# Autodesk Inventor assembly: Shooter
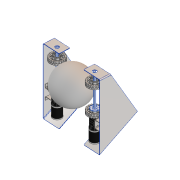
[picture p0: Inventor's stored thumbnail of the model, 180x180]
Saved by Autodesk Inventor 2016 (Build 200138000, 138)
## iProperties
Created: 2016-01-25
Part Number: Shooter
Document SubType Name: Assembly
Designer: CAD
Author: CAD
## Documents named in this file (9)
- C:\Users\PrashantBIA\Desktop\Robotics\Robot Assembly 1-27-15 New Swami\Robot Assembly\Shooter\Shooter.iam
- C:\Users\PrashantBIA\Desktop\Robotics\Robot Assembly 1-27-15 New Swami\Robot Assembly\Shooter\Imported Components\4 in HiGrip Wheel\4 in HiGrip Wheel.iam
- C:\Users\PrashantBIA\Desktop\Robotics\Robot Assembly 1-27-15 New Swami\Robot Assembly\Shooter\VersaPlanetaryWithCim.iam
- C:\Users\PrashantBIA\Desktop\Robotics\Robot Assembly 1-27-15 New Swami\Robot Assembly\Shooter\Ball.ipt
- C:\Users\PrashantBIA\Desktop\Robotics\Robot Assembly 1-27-15 New Swami\Robot Assembly\Shooter\Imported Components\am-0096a+500+Hex+Hub+r2\am-0096a+500+Hex+Hub+r2.ipt
- C:\Users\PrashantBIA\Desktop\Robotics\Robot Assembly 1-27-15 New Swami\Robot Assembly\Shooter\10inshaft.ipt
- C:\Users\PrashantBIA\Desktop\Robotics\Robot Assembly 1-27-15 New Swami\Robot Assembly\Shooter\RightMounting.ipt
- C:\Users\PrashantBIA\Desktop\Robotics\Robot Assembly 1-27-15 New Swami\Robot Assembly\Shooter\MountingForGearbox.ipt
- C:\Users\PrashantBIA\Desktop\Robotics\Robot Assembly 1-27-15 New Swami\Robot Assembly\Shooter\LeftMounting.ipt
## Components (19 placed, 8 different names)
1. VersaPlanetaryWithCim:1 [sub-assembly] — Mate:5, Flush:3, Mate:44, Flush:4, Angle:4, Angle:8, Angle:9, Mate:78, Mate:81, Mate:82
2. VersaPlanetaryWithCim:2 [sub-assembly] — Mate:2, Mate:3, Flush:3, Mate:44, Flush:4, Angle:1, Mate:52, Mate:62, Mate:84, Mate:86, Mate:87
3. Ball:1
4. 10inshaft:1 — Mate:70, Angle:7, Mate:75, Mate:76, Angle:8, Flush:8
5. 10inshaft:2 — Angle:5, Angle:6, Mate:61, Mate:62, Mate:63, Flush:9
6. RightMounting:1 — Angle:9, Mate:78, Flush:8, Mate:79
7. MountingForGearbox:1 — Mate:81, Mate:82
8. LeftMounting:1 — Mate:83, Flush:9, Mate:84, Mate:85
9. MountingForGearbox:2 — Mate:85, Mate:86, Mate:87
10. am-0096a+500+Hex+Hub+r2:1 — Mate:58, Mate:59, Mate:60, Angle:4, Mate:70
11. am-0096a+500+Hex+Hub+r2:2 — Mate:49, Mate:50, Mate:51, Angle:5, Angle:6, Mate:61, Mate:63, Flush:5, Flush:6, Mate:83
12. am-0096a+500+Hex+Hub+r2:3 — Mate:46, Mate:47, Mate:48, Angle:1, Mate:52
13. am-0096a+500+Hex+Hub+r2:4 — Mate:71, Mate:72, Mate:73, Mate:79
14. am-0096a+500+Hex+Hub+r2:5 — Mate:64, Mate:65, Mate:66, Angle:7, Mate:75, Mate:76
15. am-0096a+500+Hex+Hub+r2:7 — Mate:67, Mate:68, Mate:69, Flush:5, Flush:6
16. 4 in HiGrip Wheel:1 [sub-assembly] — Flush:1, Mate:5, Mate:58, Mate:59, Mate:60, Mate:71, Mate:72, Mate:73, Mate:74
17. 4 in HiGrip Wheel:2 [sub-assembly] — Flush:1, Mate:2, Mate:3, Mate:46, Mate:47, Mate:48, Mate:49, Mate:50, Mate:51, Mate:77
18. 4 in HiGrip Wheel:3 [sub-assembly] — Mate:64, Mate:65, Mate:66, Mate:74, Flush:7
19. 4 in HiGrip Wheel:4 [sub-assembly] — Mate:67, Mate:68, Mate:69, Mate:77, Flush:7
## Relationships (55: Mate 40, Flush 8, Angle 7)
- Flush:1: 4 in HiGrip Wheel:1 ↔ 4 in HiGrip Wheel:2
- Mate:2: VersaPlanetaryWithCim:2 ↔ 4 in HiGrip Wheel:2
- Mate:3: VersaPlanetaryWithCim:2 ↔ 4 in HiGrip Wheel:2
- Mate:5: VersaPlanetaryWithCim:1 ↔ 4 in HiGrip Wheel:1
- Flush:3: VersaPlanetaryWithCim:1 ↔ VersaPlanetaryWithCim:2
- Mate:44 (254 mm): VersaPlanetaryWithCim:1 ↔ VersaPlanetaryWithCim:2
- Flush:4: VersaPlanetaryWithCim:1 ↔ VersaPlanetaryWithCim:2
- Mate:46: am-0096a+500+Hex+Hub+r2:3 ↔ 4 in HiGrip Wheel:2
- Mate:47: am-0096a+500+Hex+Hub+r2:3 ↔ 4 in HiGrip Wheel:2
- Mate:48: am-0096a+500+Hex+Hub+r2:3 ↔ 4 in HiGrip Wheel:2
- Mate:49: am-0096a+500+Hex+Hub+r2:2 ↔ 4 in HiGrip Wheel:2
- Mate:50: am-0096a+500+Hex+Hub+r2:2 ↔ 4 in HiGrip Wheel:2
- Mate:51: am-0096a+500+Hex+Hub+r2:2 ↔ 4 in HiGrip Wheel:2
- Angle:1 (0 deg): VersaPlanetaryWithCim:2 ↔ am-0096a+500+Hex+Hub+r2:3
- Mate:52: VersaPlanetaryWithCim:2 ↔ am-0096a+500+Hex+Hub+r2:3
- Mate:58: am-0096a+500+Hex+Hub+r2:1 ↔ 4 in HiGrip Wheel:1
- Mate:59: am-0096a+500+Hex+Hub+r2:1 ↔ 4 in HiGrip Wheel:1
- Mate:60: am-0096a+500+Hex+Hub+r2:1 ↔ 4 in HiGrip Wheel:1
- Angle:4 (0 deg): VersaPlanetaryWithCim:1 ↔ am-0096a+500+Hex+Hub+r2:1
- Angle:5 (0 deg): 10inshaft:2 ↔ am-0096a+500+Hex+Hub+r2:2
- Angle:6 (0 deg): 10inshaft:2 ↔ am-0096a+500+Hex+Hub+r2:2
- Mate:61: 10inshaft:2 ↔ am-0096a+500+Hex+Hub+r2:2
- Mate:62: VersaPlanetaryWithCim:2 ↔ 10inshaft:2
- Mate:63: 10inshaft:2 ↔ am-0096a+500+Hex+Hub+r2:2
- Mate:64: am-0096a+500+Hex+Hub+r2:5 ↔ 4 in HiGrip Wheel:3
- Mate:65: am-0096a+500+Hex+Hub+r2:5 ↔ 4 in HiGrip Wheel:3
- Mate:66: am-0096a+500+Hex+Hub+r2:5 ↔ 4 in HiGrip Wheel:3
- Mate:67: am-0096a+500+Hex+Hub+r2:7 ↔ 4 in HiGrip Wheel:4
- Mate:68: am-0096a+500+Hex+Hub+r2:7 ↔ 4 in HiGrip Wheel:4
- Mate:69: am-0096a+500+Hex+Hub+r2:7 ↔ 4 in HiGrip Wheel:4
- Mate:70: 10inshaft:1 ↔ am-0096a+500+Hex+Hub+r2:1
- Mate:71: am-0096a+500+Hex+Hub+r2:4 ↔ 4 in HiGrip Wheel:1
- Mate:72: am-0096a+500+Hex+Hub+r2:4 ↔ 4 in HiGrip Wheel:1
- Mate:73: am-0096a+500+Hex+Hub+r2:4 ↔ 4 in HiGrip Wheel:1
- Mate:74: 4 in HiGrip Wheel:1 ↔ 4 in HiGrip Wheel:3
- Angle:7 (0 deg): 10inshaft:1 ↔ am-0096a+500+Hex+Hub+r2:5
- Mate:75: 10inshaft:1 ↔ am-0096a+500+Hex+Hub+r2:5
- Mate:76: 10inshaft:1 ↔ am-0096a+500+Hex+Hub+r2:5
- Angle:8 (0 deg): VersaPlanetaryWithCim:1 ↔ 10inshaft:1
- Mate:77: 4 in HiGrip Wheel:2 ↔ 4 in HiGrip Wheel:4
- Flush:5: am-0096a+500+Hex+Hub+r2:2 ↔ am-0096a+500+Hex+Hub+r2:7
- Flush:6: am-0096a+500+Hex+Hub+r2:2 ↔ am-0096a+500+Hex+Hub+r2:7
- Flush:7: 4 in HiGrip Wheel:3 ↔ 4 in HiGrip Wheel:4
- Angle:9 (0 deg): VersaPlanetaryWithCim:1 ↔ RightMounting:1
- Mate:78 (51.943 mm): VersaPlanetaryWithCim:1 ↔ RightMounting:1
- Flush:8: 10inshaft:1 ↔ RightMounting:1
- Mate:79: RightMounting:1 ↔ am-0096a+500+Hex+Hub+r2:4
- Mate:81: VersaPlanetaryWithCim:1 ↔ MountingForGearbox:1
- Mate:82: VersaPlanetaryWithCim:1 ↔ MountingForGearbox:1
- Mate:83: LeftMounting:1 ↔ am-0096a+500+Hex+Hub+r2:2
- Flush:9: 10inshaft:2 ↔ LeftMounting:1
- Mate:84 (51.943 mm): VersaPlanetaryWithCim:2 ↔ LeftMounting:1
- Mate:85: LeftMounting:1 ↔ MountingForGearbox:2
- Mate:86: VersaPlanetaryWithCim:2 ↔ MountingForGearbox:2
- Mate:87: VersaPlanetaryWithCim:2 ↔ MountingForGearbox:2
